# Autodesk Inventor assembly: Switch Assembly
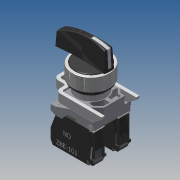
[picture p0: Inventor's stored thumbnail of the model, 180x180]
Saved by Autodesk Inventor 2014 (Build 180170000, 170)
## iProperties
Created: 2014-11-11
Part Number: Switch Assembly
Document SubType Name: Assembly
Designer: David
Author: David
## Documents named in this file (5)
- C:\Users\David\Documents\Inventor\Master\Electrical\Switches\Schneider\Switch Assembly.iam
- C:\Users\David\Documents\Inventor\Master\Electrical\Switches\Schneider\Mounting Collar.ipt
- C:\Users\David\Documents\Inventor\Master\Electrical\Switches\Schneider\Contact NC.ipt
- C:\Users\David\Documents\Inventor\Master\Electrical\Switches\Schneider\Contact NO.ipt
- C:\Users\David\Documents\Inventor\Master\Electrical\Switches\Schneider\Switch EXTENDED LEVER.ipt
## Components (4 placed, 4 different names)
1. Mounting Collar:1 — Mate:1, Flush:1, Flush:2, Mate:2, Flush:3, Flush:4, Mate:3, Mate:4
2. Contact NC:1 — Mate:1, Flush:1, Flush:2
3. Contact NO:1 — Mate:2, Flush:3, Flush:4
4. Switch EXTENDED LEVER:1 — Mate:3, Mate:4, Flush:5
## Relationships (9: Flush 5, Mate 4)
- Mate:1: Mounting Collar:1 ↔ Contact NC:1
- Flush:1: Mounting Collar:1 ↔ Contact NC:1
- Flush:2: Mounting Collar:1 ↔ Contact NC:1
- Mate:2: Mounting Collar:1 ↔ Contact NO:1
- Flush:3: Mounting Collar:1 ↔ Contact NO:1
- Flush:4: Mounting Collar:1 ↔ Contact NO:1
- Mate:3: Mounting Collar:1 ↔ Switch EXTENDED LEVER:1
- Mate:4 (6.35 mm): Mounting Collar:1 ↔ Switch EXTENDED LEVER:1
- Flush:5: Switch EXTENDED LEVER:1
